# Autodesk Inventor assembly: StangeKopfGesamptTeil
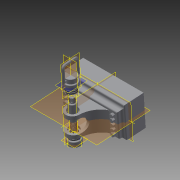
[picture p0: Inventor's stored thumbnail of the model, 180x180]
Saved by Autodesk Inventor 2015 (Build 190159000, 159)
## iProperties
Created: 2019-03-12
Part Number: StangeKopfGesamptTeil
Document SubType Name: Assembly
Designer: Boris
Author: Boris
## Documents named in this file (5)
- D:\Wisag Hiserv\HiSERV Smart Drive\WorkOrder\3D - Teile\StangeKopfGesamptTeil.iam
- D:\Wisag Hiserv\HiSERV Smart Drive\WorkOrder\3D - Teile\SchleppstangeBefestigung.ipt
- D:\Wisag Hiserv\HiSERV Smart Drive\WorkOrder\3D - Teile\SchleppstangeBefestigungOben.ipt
- D:\Wisag Hiserv\HiSERV Smart Drive\WorkOrder\3D - Teile\SchleppstangeBefestigungUnten.ipt
- D:\Wisag Hiserv\HiSERV Smart Drive\WorkOrder\3D - Teile\SchleppstangeHauptTeil.ipt
## Components (4 placed, 4 different names)
1. SchleppstangeBefestigung:1 — Einfügen:1, Einfügen:2, Einfügen:3
2. SchleppstangeBefestigungOben:1 — Einfügen:2
3. SchleppstangeBefestigungUnten:1 — Einfügen:1
4. SchleppstangeHauptTeil:1 — Einfügen:3
## Relationships (3: Insert 3)
- Einfügen:1 [Insert] (1 mm): SchleppstangeBefestigung:1 ↔ SchleppstangeBefestigungUnten:1
- Einfügen:2 [Insert] (2 mm): SchleppstangeBefestigung:1 ↔ SchleppstangeBefestigungOben:1
- Einfügen:3 [Insert]: SchleppstangeBefestigung:1 ↔ SchleppstangeHauptTeil:1
